# Autodesk Inventor assembly: tc_switchplate
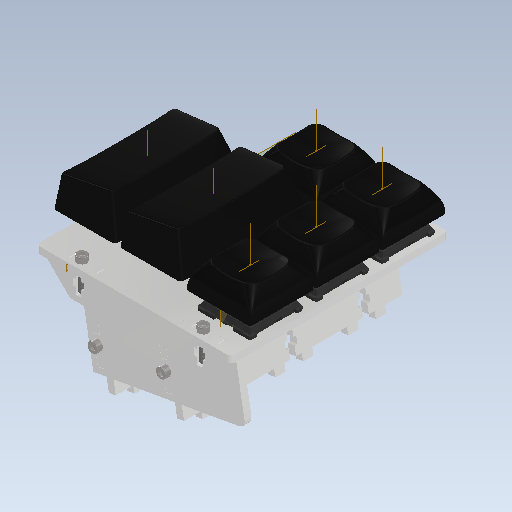
[picture p0: Inventor's stored thumbnail of the model, 512x512]
Saved by Autodesk Inventor 2020 (Build 240168000, 168)
## iProperties
Created: 2019-07-07
Part Number: tc_switchplate
Document SubType Name: Assembly
Designer: Thibault
Author: Thibault
## Documents named in this file (9)
- C:\Users\Thibault Polge\Documents\Habilis\mech\tc_switchplate.iam
- C:\Users\Thibault Polge\Documents\Habilis\mech\tc_base_plate.ipt
- C:\Users\Thibault Polge\Documents\Habilis\mech\mx\TC-R1 2×1 A.iam
- C:\Users\Thibault Polge\Documents\Habilis\mech\mx\TC-R1 2×1 B.iam
- C:\Users\Thibault Polge\Documents\Habilis\mech\mx.iam
- C:\Users\Thibault Polge\Documents\Habilis\mech\tc_support_up.ipt
- C:\Users\Thibault Polge\Documents\Habilis\mech\tc_support_down.ipt
- C:\Users\Thibault Polge\Documents\Inventor\Content Center Files\R2020\fr-FR\BS 4168(1)\BS 4168 - M1,6 x 8(1).ipt
- C:\Users\Thibault Polge\Documents\Habilis\mech\mx\DSA-1x1.iam
## Components (14 placed, 7 different names)
1. tc_base_plate:1 — Placage:1, Placage:2, Placage:3, Placage:4, Placage:5, Placage:6, Placage:7, Affleurement:1, Placage:8, Placage:9, Placage:10, Affleurement:2, Placage:11, Placage:12, Placage:13, Placage:14, Placage:15, Placage:16, Affleurement:3, Placage:17, Placage:18, Affleurement:4, Affleurement:5, Affleurement:6, Logement:3, Logement:4
2. DSA-1x1:1 [sub-assembly] — Placage:4, Placage:9, Placage:15
3. DSA-1x1:2 [sub-assembly] — Placage:2, Affleurement:1, Placage:12
4. DSA-1x1:3 [sub-assembly] — Placage:5, Placage:10, Placage:16
5. TC-R1 2×1 A:4 [sub-assembly] — Placage:3, Placage:7, Placage:13
6. TC-R1 2×1 B:5 [sub-assembly] — Placage:6, Affleurement:2, Placage:14
7. DSA-1x1:6 [sub-assembly] — Placage:1, Placage:8, Placage:11
8. tc_support_up:1 — Affleurement:3, Placage:17, Placage:18, Affleurement:7, Placage:19, Placage:20, Affleurement:8, Placage:21, Placage:22, Logement:1, Logement:2
9. tc_support_down:1 — Affleurement:7, Placage:19, Placage:20
10. tc_support_down:2 — Affleurement:8, Placage:21, Placage:22
11. BS 4168 : Pièce 1 Vis cylindrique à six pans creux - Métrique M1,6 x 8:1 — Logement:1
12. BS 4168 : Pièce 1 Vis cylindrique à six pans creux - Métrique M1,6 x 8:2 — Logement:2
13. BS 4168 : Pièce 1 Vis cylindrique à six pans creux - Métrique M1,6 x 8:3 — Logement:3
14. BS 4168 : Pièce 1 Vis cylindrique à six pans creux - Métrique M1,6 x 8:4 — Logement:4
## Relationships (34: Mate 22, Flush 8, Insert 4)
- Placage:1 [Mate]: tc_base_plate:1 ↔ DSA-1x1:6
- Placage:2 [Mate]: tc_base_plate:1 ↔ DSA-1x1:2
- Placage:3 [Mate]: tc_base_plate:1 ↔ TC-R1 2×1 A:4
- Placage:4 [Mate]: tc_base_plate:1 ↔ DSA-1x1:1
- Placage:5 [Mate]: tc_base_plate:1 ↔ DSA-1x1:3
- Placage:6 [Mate]: tc_base_plate:1 ↔ TC-R1 2×1 B:5
- Placage:7 [Mate]: tc_base_plate:1 ↔ TC-R1 2×1 A:4
- Affleurement:1 [Flush]: tc_base_plate:1 ↔ DSA-1x1:2
- Placage:8 [Mate]: tc_base_plate:1 ↔ DSA-1x1:6
- Placage:9 [Mate]: tc_base_plate:1 ↔ DSA-1x1:1
- Placage:10 [Mate]: tc_base_plate:1 ↔ DSA-1x1:3
- Affleurement:2 [Flush]: tc_base_plate:1 ↔ TC-R1 2×1 B:5
- Placage:11 [Mate]: tc_base_plate:1 ↔ DSA-1x1:6
- Placage:12 [Mate]: tc_base_plate:1 ↔ DSA-1x1:2
- Placage:13 [Mate]: tc_base_plate:1 ↔ TC-R1 2×1 A:4
- Placage:14 [Mate]: tc_base_plate:1 ↔ TC-R1 2×1 B:5
- Placage:15 [Mate]: tc_base_plate:1 ↔ DSA-1x1:1
- Placage:16 [Mate]: tc_base_plate:1 ↔ DSA-1x1:3
- Affleurement:3 [Flush]: tc_base_plate:1 ↔ tc_support_up:1
- Placage:17 [Mate]: tc_base_plate:1 ↔ tc_support_up:1
- Placage:18 [Mate]: tc_base_plate:1 ↔ tc_support_up:1
- Affleurement:4 [Flush]: tc_base_plate:1
- Affleurement:5 [Flush]: tc_base_plate:1
- Affleurement:6 [Flush]: tc_base_plate:1
- Affleurement:7 [Flush]: tc_support_up:1 ↔ tc_support_down:1
- Placage:19 [Mate]: tc_support_up:1 ↔ tc_support_down:1
- Placage:20 [Mate]: tc_support_up:1 ↔ tc_support_down:1
- Affleurement:8 [Flush]: tc_support_up:1 ↔ tc_support_down:2
- Placage:21 [Mate]: tc_support_up:1 ↔ tc_support_down:2
- Placage:22 [Mate]: tc_support_up:1 ↔ tc_support_down:2
- Logement:1 [Insert]: tc_support_up:1 ↔ BS 4168 : Pièce 1 Vis cylindrique à six pans creux - Métrique M1,6 x 8:1
- Logement:2 [Insert]: tc_support_up:1 ↔ BS 4168 : Pièce 1 Vis cylindrique à six pans creux - Métrique M1,6 x 8:2
- Logement:3 [Insert]: tc_base_plate:1 ↔ BS 4168 : Pièce 1 Vis cylindrique à six pans creux - Métrique M1,6 x 8:3
- Logement:4 [Insert]: tc_base_plate:1 ↔ BS 4168 : Pièce 1 Vis cylindrique à six pans creux - Métrique M1,6 x 8:4
